# Autodesk Inventor assembly: RaspberryPi
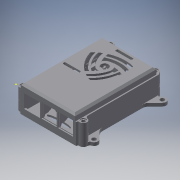
[picture p0: Inventor's stored thumbnail of the model, 180x180]
Saved by Autodesk Inventor 2019 (Build 230136000, 136)
## iProperties
Created: 2019-12-10
Part Number: RaspberryPi
Document SubType Name: Assembly
Designer: james
Author: james
## Documents named in this file (3)
- F:\JimsRobot\FIRSTRobots\Design\Library\Jims\RaspberryPi.iam
- F:\JimsRobot\FIRSTRobots\Design\Library\Jims\rpi2-bottom.ipt
- F:\JimsRobot\FIRSTRobots\Design\Library\Jims\rpi2-top.ipt
## Components (2 placed, 2 different names)
1. rpi2-bottom:1 — Mate:1, Mate:2, Mate:3
2. rpi2-top:1 — Mate:1, Mate:2, Mate:3
## Relationships (3: Mate 3)
- Mate:1: rpi2-bottom:1 ↔ rpi2-top:1
- Mate:2: rpi2-bottom:1 ↔ rpi2-top:1
- Mate:3: rpi2-bottom:1 ↔ rpi2-top:1
